# Autodesk Inventor assembly: gripper assembly
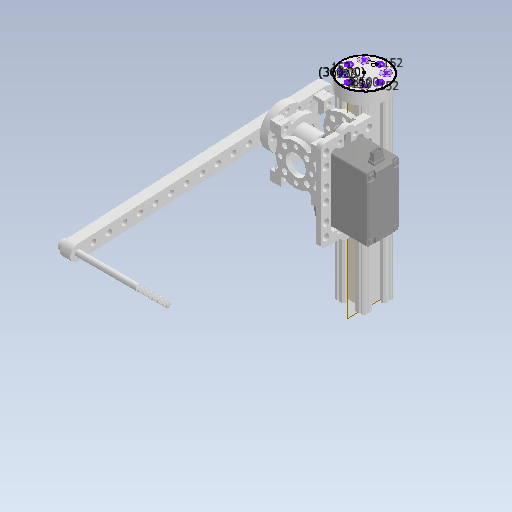
[picture p0: Inventor's stored thumbnail of the model, 512x512]
Saved by Autodesk Inventor 2020 (Build 240168000, 168)
## iProperties
Created: 2020-01-03
Part Number: gripper assembly
Document SubType Name: Assembly
Designer: ball
Author: ball
## Documents named in this file (6)
- D:\FTC8863\2019 Robot\Collection\gripper assembly.iam
- D:\FTC8863\Actobotics\565 parts\565026.ipt
- D:\FTC8863\2019 Robot\Collection\servo block assembly.iam
- D:\FTC8863\2019 Robot\Collection\grabber arm.ipt
- D:\FTC8863\StepLibraries\Screws\92196A161_18-8 STAINLESS STEEL SOCKET HEAD CAP SCREW (1).ipt
- D:\FTC8863\2019 Robot\Collection\Collector rotation xrail to turntable adapter.ipt
## Components (5 placed, 5 different names)
1. 565026:1 — Mate:1, Mate:2, Mate:3, Flush:1, Mate:11, Mate:12, Mate:13
2. servo block assembly:1 [sub-assembly] — Mate:1, Mate:2, Mate:3, Flush:1, Mate:4, Mate:5, Mate:6
3. grabber arm:1 — Mate:4, Mate:5, Mate:6, Mate:7, Mate:8
4. 92196A161_18-8 STAINLESS STEEL SOCKET HEAD CAP SCREW (1):1 — Mate:7, Mate:8
5. Collector rotation xrail to turntable adapter:1 — Mate:11, Mate:12, Mate:13
## Relationships (12: Mate 11, Flush 1)
- Mate:1: 565026:1 ↔ servo block assembly:1
- Mate:2: 565026:1 ↔ servo block assembly:1
- Mate:3: 565026:1 ↔ servo block assembly:1
- Flush:1 (77.216 mm): 565026:1 ↔ servo block assembly:1
- Mate:4: servo block assembly:1 ↔ grabber arm:1
- Mate:5: servo block assembly:1 ↔ grabber arm:1
- Mate:6: servo block assembly:1 ↔ grabber arm:1
- Mate:7: grabber arm:1 ↔ 92196A161_18-8 STAINLESS STEEL SOCKET HEAD CAP SCREW (1):1
- Mate:8: grabber arm:1 ↔ 92196A161_18-8 STAINLESS STEEL SOCKET HEAD CAP SCREW (1):1
- Mate:11: 565026:1 ↔ Collector rotation xrail to turntable adapter:1
- Mate:12: 565026:1 ↔ Collector rotation xrail to turntable adapter:1
- Mate:13: 565026:1 ↔ Collector rotation xrail to turntable adapter:1
